# Autodesk Inventor assembly: X_CarriageR_V2_0
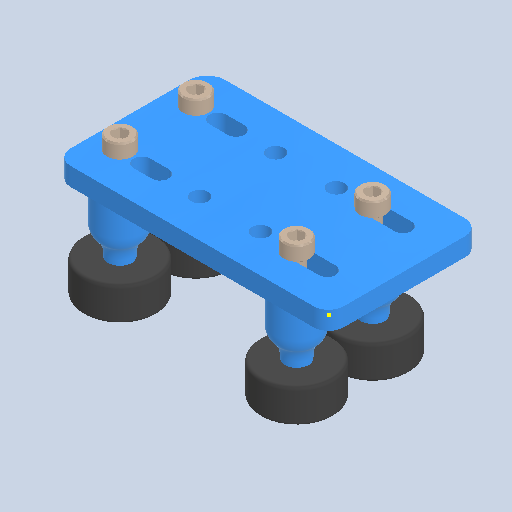
[picture p0: Inventor's stored thumbnail of the model, 512x512]
Saved by Autodesk Inventor 2022 (Build 260153000, 153)
## iProperties
Created: 2021-06-13
Part Number: X_CarriageR_V2_0
Document SubType Name: Assembly
Designer: Jorian Brusind
Author: Jorian Brusind
## Documents named in this file (7)
- C:\Users\Jorian Brusind\Documents\GitHub\HyperRail\Inventor Files\X_CarriageR_V2_0.iam
- C:\Users\Jorian Brusind\Documents\GitHub\HyperRail\Inventor Files\X_Carriage_Plate.ipt
- C:\Users\Jorian Brusind\Documents\GitHub\HyperRail\Inventor Files\11mm_BearingWheel.ipt
- C:\Users\Jorian Brusind\Documents\GitHub\HyperRail\Inventor Files\4mm_Roller_Spacer_simple.ipt
- C:\Users\Jorian Brusind\Documents\GitHub\HyperRail\Inventor Files\Metric Spacer_Standoffs\hex spacer standoff nut M5 L30.ipt
- C:\Users\Jorian Brusind\Documents\GitHub\HyperRail\Inventor Files\Metric bolt\Bolt M5 30mm.ipt
- C:\Users\Jorian Brusind\Documents\GitHub\HyperRail\Inventor Files\Metric bolt\Bolt M5 45mm.ipt
## Components (14 placed, 6 different names)
1. X_Carriage_Plate:1 — Mate:13, Mate:57, Mate:60, Angle:1, Angle:2, Mate:63, Mate:77
2. 11mm_BearingWheel:1 — Flush:2, Mate:62
3. 11mm_BearingWheel:4 — Flush:2, Mate:58, Mate:61
4. 4mm_Roller_Spacer_simple:1 — Mate:13, Mate:60, Angle:1, Mate:64, Mate:65, Mate:66, Mate:67, Mate:70, Mate:71, Mate:73, Mate:74
5. 4mm_Roller_Spacer_simple:2 — Mate:57, Mate:58, Mate:61, Mate:62, Angle:2, Mate:63, Mate:68, Mate:69, Mate:72, Mate:75, Mate:76
6. 11mm_BearingWheel:5 — Mate:64, Flush:3
7. 11mm_BearingWheel:6 — Mate:65, Flush:3, Mate:66
8. hex spacer standoff nut M5 L30:1 — Mate:67, Mate:68
9. Bolt M5 30mm:1 — Mate:69, Mate:72
10. Bolt M5 30mm:2 — Mate:70, Mate:71
11. Bolt M5 45mm:1 — Mate:74, Flush:5, Flush:6
12. Bolt M5 45mm:2 — Mate:73, Flush:4, Flush:5
13. Bolt M5 45mm:3 — Mate:76, Flush:6, Mate:77
14. Bolt M5 45mm:4 — Mate:75, Flush:4
## Relationships (28: Mate 21, Flush 5, Angle 2)
- Flush:2: 11mm_BearingWheel:1 ↔ 11mm_BearingWheel:4
- Mate:13: X_Carriage_Plate:1 ↔ 4mm_Roller_Spacer_simple:1
- Mate:57: X_Carriage_Plate:1 ↔ 4mm_Roller_Spacer_simple:2
- Mate:58: 11mm_BearingWheel:4 ↔ 4mm_Roller_Spacer_simple:2
- Mate:60 (-12.5 mm): X_Carriage_Plate:1 ↔ 4mm_Roller_Spacer_simple:1
- Angle:1 (0 deg): X_Carriage_Plate:1 ↔ 4mm_Roller_Spacer_simple:1
- Mate:61: 11mm_BearingWheel:4 ↔ 4mm_Roller_Spacer_simple:2
- Mate:62: 11mm_BearingWheel:1 ↔ 4mm_Roller_Spacer_simple:2
- Angle:2 (0 deg): X_Carriage_Plate:1 ↔ 4mm_Roller_Spacer_simple:2
- Mate:63 (-12.5 mm): X_Carriage_Plate:1 ↔ 4mm_Roller_Spacer_simple:2
- Mate:64: 4mm_Roller_Spacer_simple:1 ↔ 11mm_BearingWheel:5
- Mate:65: 4mm_Roller_Spacer_simple:1 ↔ 11mm_BearingWheel:6
- Flush:3: 11mm_BearingWheel:5 ↔ 11mm_BearingWheel:6
- Mate:66: 4mm_Roller_Spacer_simple:1 ↔ 11mm_BearingWheel:6
- Mate:67: 4mm_Roller_Spacer_simple:1 ↔ hex spacer standoff nut M5 L30:1
- Mate:68 (5 mm): 4mm_Roller_Spacer_simple:2 ↔ hex spacer standoff nut M5 L30:1
- Mate:69: 4mm_Roller_Spacer_simple:2 ↔ Bolt M5 30mm:1
- Mate:70: 4mm_Roller_Spacer_simple:1 ↔ Bolt M5 30mm:2
- Mate:71: 4mm_Roller_Spacer_simple:1 ↔ Bolt M5 30mm:2
- Mate:72: 4mm_Roller_Spacer_simple:2 ↔ Bolt M5 30mm:1
- Mate:73: 4mm_Roller_Spacer_simple:1 ↔ Bolt M5 45mm:2
- Mate:74: 4mm_Roller_Spacer_simple:1 ↔ Bolt M5 45mm:1
- Mate:75: 4mm_Roller_Spacer_simple:2 ↔ Bolt M5 45mm:4
- Mate:76: 4mm_Roller_Spacer_simple:2 ↔ Bolt M5 45mm:3
- Flush:4: Bolt M5 45mm:2 ↔ Bolt M5 45mm:4
- Flush:5: Bolt M5 45mm:1 ↔ Bolt M5 45mm:2
- Flush:6: Bolt M5 45mm:1 ↔ Bolt M5 45mm:3
- Mate:77: X_Carriage_Plate:1 ↔ Bolt M5 45mm:3
